# Autodesk Inventor assembly: total_model
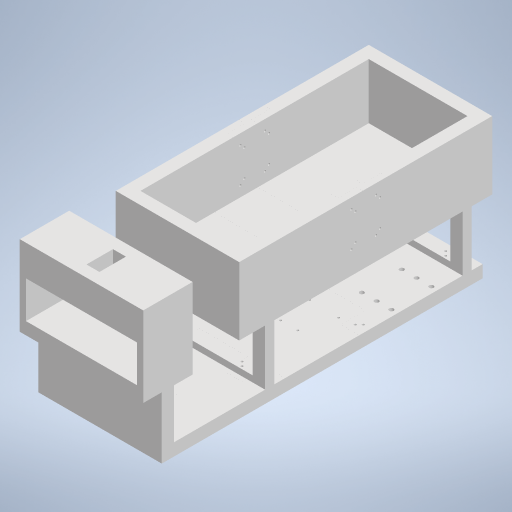
[picture p0: Inventor's stored thumbnail of the model, 512x512]
Saved by Autodesk Inventor 2023 (Build 270158000, 158)
## iProperties
Created: 2022-11-29
Part Number: total_model
Document SubType Name: Assembly
Designer: inigo
Author: inigo
## Documents named in this file (8)
- D:\projects\FoBo\model\total_model.iam
- D:\projects\FoBo\model\base_back.ipt
- D:\projects\FoBo\model\base_front.ipt
- D:\projects\FoBo\model\base_mid.ipt
- D:\projects\FoBo\model\front_support.ipt
- D:\projects\FoBo\model\container_front.ipt
- D:\projects\FoBo\model\container_back.ipt
- D:\projects\FoBo\model\container_mid.ipt
## Components (7 placed, 7 different names)
1. base_back:1 — Coincidencia:4, Coincidencia:5, Coincidencia:6, Coincidencia:12
2. base_front:1 — Coincidencia:1, Coincidencia:2, Coincidencia:3, Coincidencia:7, Coincidencia:8, Coincidencia:9, Coincidencia:13
3. base_mid:1 — Coincidencia:1, Coincidencia:2, Coincidencia:3, Coincidencia:4, Coincidencia:5, Coincidencia:6
4. front_support:1 — Coincidencia:7, Coincidencia:8, Coincidencia:9
5. container_front:1 — Nivelación:1, Nivelación:2, Coincidencia:10, Nivelación:3, Nivelación:4, Coincidencia:13
6. container_mid:1 — Nivelación:1, Nivelación:2, Coincidencia:10, Coincidencia:11
7. container_back:1 — Nivelación:3, Nivelación:4, Coincidencia:11, Coincidencia:12
## Relationships (17: Mate 13, Flush 4)
- Coincidencia:1 [Mate]: base_front:1 ↔ base_mid:1
- Coincidencia:2 [Mate]: base_front:1 ↔ base_mid:1
- Coincidencia:3 [Mate]: base_front:1 ↔ base_mid:1
- Coincidencia:4 [Mate]: base_back:1 ↔ base_mid:1
- Coincidencia:5 [Mate]: base_back:1 ↔ base_mid:1
- Coincidencia:6 [Mate]: base_back:1 ↔ base_mid:1
- Coincidencia:7 [Mate]: base_front:1 ↔ front_support:1
- Coincidencia:8 [Mate]: base_front:1 ↔ front_support:1
- Coincidencia:9 [Mate]: base_front:1 ↔ front_support:1
- Nivelación:1 [Flush]: container_front:1 ↔ container_mid:1
- Nivelación:2 [Flush]: container_front:1 ↔ container_mid:1
- Coincidencia:10 [Mate]: container_front:1 ↔ container_mid:1
- Nivelación:3 [Flush]: container_front:1 ↔ container_back:1
- Nivelación:4 [Flush]: container_front:1 ↔ container_back:1
- Coincidencia:11 [Mate]: container_mid:1 ↔ container_back:1
- Coincidencia:12 [Mate]: base_back:1 ↔ container_back:1
- Coincidencia:13 [Mate]: base_front:1 ↔ container_front:1
